# Autodesk Inventor assembly: Coil Designs
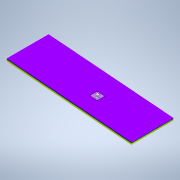
[picture p0: Inventor's stored thumbnail of the model, 180x180]
Saved by Autodesk Inventor 2021 (Build 250183000, 183)
## iProperties
Created: 2022-01-19
Part Number: Coil Designs
Document SubType Name: Assembly
Designer: avan411
Author: avan411
## Documents named in this file (9)
- \\unifiles.uoa.auckland.ac.nz\myhome\Documents\GitHub\2021_SRW_RC_CAR\Magnetics\Final Coil Design\CadModels\Coil Designs.iam
- \\unifiles.uoa.auckland.ac.nz\myhome\Documents\GitHub\2021_SRW_RC_CAR\Magnetics\Final Coil Design\CadModels\Part2.ipt
- \\unifiles.uoa.auckland.ac.nz\myhome\Documents\GitHub\2021_SRW_RC_CAR\Magnetics\Final Coil Design\CadModels\PrimaryCoilFerriteLayer.ipt
- \\unifiles.uoa.auckland.ac.nz\myhome\Documents\GitHub\2021_SRW_RC_CAR\Magnetics\Final Coil Design\CadModels\btwnFerriteAndCoil.ipt
- \\unifiles.uoa.auckland.ac.nz\myhome\Documents\GitHub\2021_SRW_RC_CAR\Magnetics\Final Coil Design\CadModels\between aluminium and ferrite.ipt
- \\unifiles.uoa.auckland.ac.nz\myhome\Documents\GitHub\2021_SRW_RC_CAR\Magnetics\Final Coil Design\CadModels\PrimaryCoilAluminiumLayer.ipt
- \\unifiles.uoa.auckland.ac.nz\myhome\Documents\GitHub\2021_SRW_RC_CAR\Magnetics\Final Coil Design\CadModels\aluminium.ipt
- \\unifiles.uoa.auckland.ac.nz\myhome\Documents\GitHub\2021_SRW_RC_CAR\Magnetics\Final Coil Design\CadModels\base.ipt
- \\unifiles.uoa.auckland.ac.nz\myhome\Documents\GitHub\2021_SRW_RC_CAR\Magnetics\Final Coil Design\CadModels\coil.ipt
## Components (8 placed, 8 different names)
1. PrimaryCoilLayer:1
2. btwnFerriteAndCoil:1 — Mate:3
3. PrimaryCoifERRITElLayer:2 — Mate:3, Flush:6
4. between aluminium and ferrite:1 — Flush:6, Flush:7, Flush:8, Mate:4, Flush:9, Flush:10
5. PrimaryCoiAluminiumlLayer:3 — Flush:7, Flush:8, Mate:4, Flush:11, Flush:12, Mate:5
6. aluminium:1 — Flush:9, Flush:10
7. base:1 — Flush:11, Flush:12, Mate:5
8. coil:1
## Relationships (10: Flush 7, Mate 3)
- Mate:3: btwnFerriteAndCoil:1 ↔ PrimaryCoifERRITElLayer:2
- Flush:6: PrimaryCoifERRITElLayer:2 ↔ between aluminium and ferrite:1
- Flush:7: between aluminium and ferrite:1 ↔ PrimaryCoiAluminiumlLayer:3
- Flush:8: between aluminium and ferrite:1 ↔ PrimaryCoiAluminiumlLayer:3
- Mate:4: between aluminium and ferrite:1 ↔ PrimaryCoiAluminiumlLayer:3
- Flush:9: between aluminium and ferrite:1 ↔ aluminium:1
- Flush:10: between aluminium and ferrite:1 ↔ aluminium:1
- Flush:11: PrimaryCoiAluminiumlLayer:3 ↔ base:1
- Flush:12: PrimaryCoiAluminiumlLayer:3 ↔ base:1
- Mate:5: PrimaryCoiAluminiumlLayer:3 ↔ base:1
